# Autodesk Inventor assembly: Assembled_Cutter
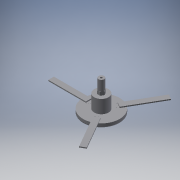
[picture p0: Inventor's stored thumbnail of the model, 180x180]
Saved by Autodesk Inventor 2019 (Build 230136000, 136)
## iProperties
Created: 2019-03-03
Part Number: Assembled_Cutter
Document SubType Name: Assembly
Designer: alarr
Author: alarr
## Documents named in this file (3)
- C:\Users\alarr\OneDrive\Documents\Inventor\Mr.Green\Assembled_Cutter.iam
- C:\Users\alarr\OneDrive\Documents\Inventor\Mr.Green\Cutter.ipt
- C:\Users\alarr\OneDrive\Documents\Inventor\Mr.Green\Cutting_Cable.ipt
## Components (2 placed, 2 different names)
1. Cutter:1 — Flush:1, Mate:1, Angle:1, Flush:2
2. Cutting_Cable:1 — Flush:2
## Relationships (4: Flush 2, Mate 1, Angle 1)
- Flush:1: Cutter:1
- Mate:1: Cutter:1
- Angle:1 (0 deg): Cutter:1
- Flush:2: Cutter:1 ↔ Cutting_Cable:1
